# Autodesk Inventor assembly: 装配体2
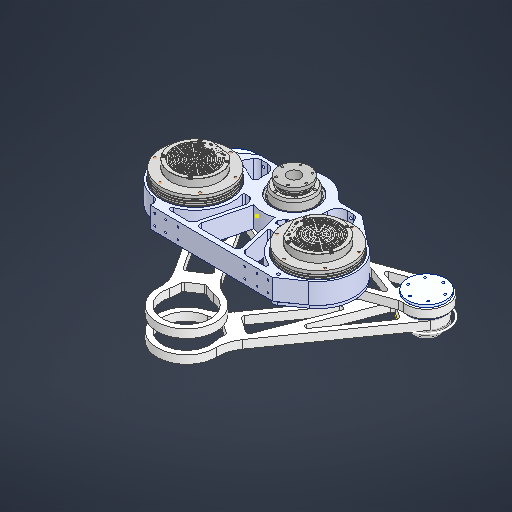
[picture p0: Inventor's stored thumbnail of the model, 512x512]
Saved by Autodesk Inventor 2025 (Build 290162000, 162)
## iProperties
Created: 2025-03-28
Part Number: 装配体2
Document SubType Name: Assembly
Designer: XH
Sending System: SolidWorks 2018
Last Author: Standard
Last Saved: 2025-04-01
代号代码: Assembly.Extension.CustomPropertyManager("").Set("代号",Left(Assembly.GetTitle,InStr(Assembly.GetTitle," ")-1))
名称代码: Assembly.Extension.CustomPropertyManager("").Set("名称",Right(Assembly.GetTitle,Len(Assembly.GetTitle)-InStr(Assembly.GetTitle," ")))
日期: 1800-01-01
名称: 装配体2
Weight: 12.94
版本号: a.1
图样标记S: S
基本计量单位（必填）: 个
Author: XH
## Documents named in this file (18)
- C:\1A_Engineering_files\RCInventor并联腿\装配体2.iam
- C:\1A_Engineering_files\RCInventor并联腿\零件6.ipt
- C:\1A_Engineering_files\RCInventor并联腿\零件7.ipt
- C:\1A_Engineering_files\RCInventor并联腿\BAR6806.ipt
- C:\1A_Engineering_files\RCInventor并联腿\零件1.ipt
- C:\1A_Engineering_files\RCInventor并联腿\61810.ipt
- C:\1A_Engineering_files\RCInventor并联腿\2.ipt
- C:\1A_Engineering_files\RCInventor并联腿\零件4.ipt
- C:\1A_Engineering_files\RCInventor并联腿\31231.ipt
- C:\1A_Engineering_files\RCInventor并联腿\零件54848.ipt
- C:\1A_Engineering_files\RCInventor并联腿\碗组\标件_碗组总成.iam
- C:\1A_Engineering_files\RCInventor并联腿\碗组\机加工_碗组连接1.ipt
- C:\1A_Engineering_files\RCInventor并联腿\碗组\碗组_培林总成.ipt
- C:\1A_Engineering_files\RCInventor并联腿\碗组\碗组_下底.ipt
- C:\1A_Engineering_files\RCInventor并联腿\碗组\板材_垫块.ipt
- C:\1A_Engineering_files\RCInventor并联腿\机加件-髋关节复合固定件.ipt
- C:\1A_Engineering_files\RCInventor并联腿\碳纤维(cnc)-关节电机端子延展固定.ipt
- C:\1A_Engineering_files\RCInventor并联腿\dm8009-20240822.iam
## Components (26 placed, 17 different names)
1. 零件6:1 — 配合:8, 配合:20, 配合:43, 配合:44, 配合:45, 配合:47, 配合:53
2. 零件7:1
3. BAR6806:1 — 配合:47, 配合:51, 配合:53
4. 零件1:1 — 配合:45, 配合:46, 配合:48, 配合:49, 配合:51, 配合:52, 配合:56, 配合:59
5. BAR6806:2 — 配合:43, 配合:52
6. 61810:1 — 配合:44, 配合:58
7. 61810:2 — 配合:46, 配合:57, 配合:59
8. 2:1 — 配合:34, 配合:35, 配合:36, 配合:48, 配合:49
9. 零件4:1 — 配合:5, 配合:8, 配合:9, 配合:20, 配合:63, 配合:64
10. 31231:1 — 配合:21, 配合:27, 配合:32, 配合:33, 配合:69
11. 零件54848:1
12. 标件_碗组总成:1 [sub-assembly] — 配合:5, 配合:10, 配合:62, 配合:63
13. 机加工_碗组连接1:1 — 配合:9, 配合:10, 配合:17, 配合:65, 配合:68
14. 碗组_培林总成:1 — 配合:12, 配合:13, 配合:62, 配合:64
15. 碗组_下底:1 — 配合:12, 配合:13
16. 板材_垫块:1 — 配合:17, 配合:66, 配合:67
17. 标件_碗组总成:2 [sub-assembly] — 配合:21, 配合:27, 配合:37
18. 机加工_碗组连接1:2 — 配合:31, 配合:35, 配合:36, 配合:37
19. 碗组_培林总成:2 — 配合:31, 配合:32, 配合:33
20. 碗组_下底:2
21. 板材_垫块:2 — 配合:34
22. 机加件-髋关节复合固定件:1 — 配合:38, 配合:39, 配合:40, 配合:42, 配合:54, 配合:55, 配合:56, 配合:57, 配合:58
23. 碳纤维(cnc)-关节电机端子延展固定:1 — 配合:38, 配合:39, 配合:40, 配合:41
24. dm8009-20240822:1 [sub-assembly] — 配合:41, 配合:42
25. dm8009-20240822:2 [sub-assembly] — 配合:54, 配合:55
26. 31231:2 — 配合:65, 配合:66, 配合:67, 配合:68, 配合:69
## Relationships (49: Mate 49)
- 配合:5 [Mate]: 零件4:1 ↔ 标件_碗组总成:1
- 配合:8 [Mate]: 零件6:1 ↔ 零件4:1
- 配合:9 [Mate]: 零件4:1 ↔ 机加工_碗组连接1:1
- 配合:10 [Mate]: 标件_碗组总成:1 ↔ 机加工_碗组连接1:1
- 配合:12 [Mate]: 碗组_培林总成:1 ↔ 碗组_下底:1
- 配合:13 [Mate]: 碗组_培林总成:1 ↔ 碗组_下底:1
- 配合:17 [Mate]: 机加工_碗组连接1:1 ↔ 板材_垫块:1
- 配合:20 [Mate]: 零件6:1 ↔ 零件4:1
- 配合:21 [Mate]: 31231:1 ↔ 标件_碗组总成:2
- 配合:27 [Mate]: 31231:1 ↔ 标件_碗组总成:2
- [Mate]: 碗组_培林总成:2 ↔ 碗组_下底:2
- [Mate]: 碗组_培林总成:2 ↔ 碗组_下底:2
- [Mate]: 机加工_碗组连接1:2 ↔ 板材_垫块:2
- 配合:31 [Mate]: 机加工_碗组连接1:2 ↔ 碗组_培林总成:2
- 配合:32 [Mate]: 31231:1 ↔ 碗组_培林总成:2
- 配合:33 [Mate]: 31231:1 ↔ 碗组_培林总成:2
- 配合:34 [Mate]: 2:1 ↔ 板材_垫块:2
- 配合:35 [Mate]: 2:1 ↔ 机加工_碗组连接1:2
- 配合:36 [Mate]: 2:1 ↔ 机加工_碗组连接1:2
- 配合:37 [Mate]: 标件_碗组总成:2 ↔ 机加工_碗组连接1:2
- 配合:38 [Mate]: 机加件-髋关节复合固定件:1 ↔ 碳纤维(cnc)-关节电机端子延展固定:1
- 配合:39 [Mate]: 机加件-髋关节复合固定件:1 ↔ 碳纤维(cnc)-关节电机端子延展固定:1
- 配合:40 [Mate]: 机加件-髋关节复合固定件:1 ↔ 碳纤维(cnc)-关节电机端子延展固定:1
- 配合:41 [Mate]: 碳纤维(cnc)-关节电机端子延展固定:1 ↔ dm8009-20240822:1
- 配合:42 [Mate]: 机加件-髋关节复合固定件:1 ↔ dm8009-20240822:1
- 配合:43 [Mate]: 零件6:1 ↔ BAR6806:2
- 配合:44 [Mate]: 零件6:1 ↔ 61810:1
- 配合:45 [Mate]: 零件6:1 ↔ 零件1:1
- 配合:46 [Mate]: 零件1:1 ↔ 61810:2
- 配合:47 [Mate]: 零件6:1 ↔ BAR6806:1
- 配合:48 [Mate]: 零件1:1 ↔ 2:1
- 配合:49 [Mate]: 零件1:1 ↔ 2:1
- 配合:51 [Mate]: BAR6806:1 ↔ 零件1:1
- 配合:52 [Mate]: 零件1:1 ↔ BAR6806:2
- 配合:53 [Mate]: 零件6:1 ↔ BAR6806:1
- 配合:54 [Mate]: 机加件-髋关节复合固定件:1 ↔ dm8009-20240822:2
- 配合:55 [Mate]: 机加件-髋关节复合固定件:1 ↔ dm8009-20240822:2
- 配合:56 [Mate]: 零件1:1 ↔ 机加件-髋关节复合固定件:1
- 配合:57 [Mate]: 61810:2 ↔ 机加件-髋关节复合固定件:1
- 配合:58 [Mate]: 61810:1 ↔ 机加件-髋关节复合固定件:1
- 配合:59 [Mate]: 零件1:1 ↔ 61810:2
- 配合:62 [Mate]: 标件_碗组总成:1 ↔ 碗组_培林总成:1
- 配合:63 [Mate]: 零件4:1 ↔ 标件_碗组总成:1
- 配合:64 [Mate]: 零件4:1 ↔ 碗组_培林总成:1
- 配合:65 [Mate]: 机加工_碗组连接1:1 ↔ 31231:2
- 配合:66 [Mate]: 板材_垫块:1 ↔ 31231:2
- 配合:67 [Mate]: 板材_垫块:1 ↔ 31231:2
- 配合:68 [Mate]: 机加工_碗组连接1:1 ↔ 31231:2
- 配合:69 [Mate]: 31231:1 ↔ 31231:2
## Named parameters: d27_d11 = 0 mm, d28_d12 = 0 mm, d29_d16 = 0 mm
